# Autodesk Inventor assembly: SEPARACION LATA-BOTELLA Y PAPEL
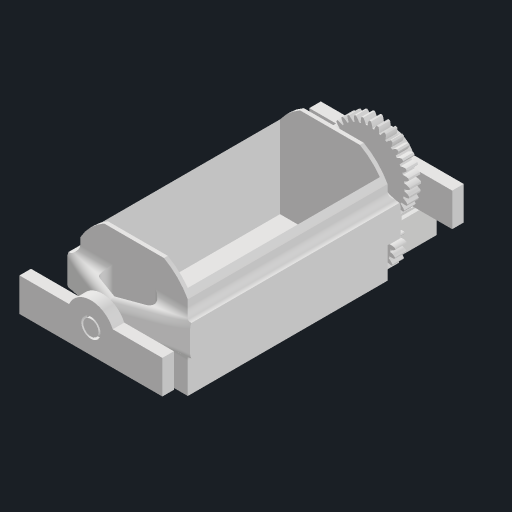
[picture p0: Inventor's stored thumbnail of the model, 512x512]
Saved by Autodesk Inventor 2024.3 (Build 283343000, 343)
## iProperties
Created: 2024-06-16
Part Number: SEPARACION LATA-BOTELLA Y PAPEL
Document SubType Name: Assembly
Designer: Jhuliams
Author: Jhuliams
## Documents named in this file (7)
- C:\Users\Niler\OneDrive\Escritorio\RECICLADOR\RECICLADOR_MODELO_3D\MECANISMO DE COMPACTADO\SEPARACION LATA-BOTELLA Y PAPEL.iam
- C:\Users\Niler\OneDrive\Escritorio\RECICLADOR\RECICLADOR_MODELO_3D\MECANISMO DE COMPACTADO\CAJA PARA DETECCION DE OBJETO.ipt
- C:\Users\Niler\OneDrive\Escritorio\RECICLADOR\RECICLADOR_MODELO_3D\MECANISMO DE COMPACTADO\ENGRANAJE CONDUCTOR DE CAJA.ipt
- C:\Users\Niler\OneDrive\Escritorio\RECICLADOR\RECICLADOR_MODELO_3D\MECANISMO DE COMPACTADO\ENGRANE MOTRIZ DE CAJA.ipt
- C:\Users\Niler\OneDrive\Escritorio\RECICLADOR\RECICLADOR_MODELO_3D\MECANISMO DE COMPACTADO\SOPORTE DE CAJA SEPARADORA.ipt
- C:\Users\Niler\OneDrive\Escritorio\RECICLADOR\RECICLADOR_MODELO_3D\MECANISMO DE COMPACTADO\NEMA 17 PARA TAPA PRINCIPAL.ipt
- C:\Users\Niler\OneDrive\Escritorio\RECICLADOR\RECICLADOR_MODELO_3D\MECANISMO DE COMPACTADO\SOPORTE DE NEMA.ipt
## Components (7 placed, 6 different names)
1. CAJA PARA DETECCION DE OBJETO:1 — Mate:3, Mate:4, Flush:2, Mate:5, Flush:3, Flush:6, Mate:9, Flush:7
2. ENGRANAJE CONDUCTOR DE CAJA:1 — Flush:1, Mate:2, Mate:3, Rotation:1, Mate:9
3. ENGRANE MOTRIZ DE CAJA:1 — Flush:1, Mate:2, Rotation:1, Mate:6, Flush:5
4. SOPORTE DE CAJA SEPARADORA:1 — Mate:5, Flush:3, Flush:6
5. SOPORTE DE CAJA SEPARADORA:2 — Mate:4, Flush:2, Flush:7
6. NEMA 17 PARA TAPA PRINCIPAL:1 — Mate:6, Flush:5, Mate:7, Mate:8, Flush:8
7. SOPORTE DE NEMA:1 — Mate:7, Mate:8, Flush:8
## Relationships (16: Mate 8, Flush 7, RelateRotation 1)
- Flush:1: ENGRANAJE CONDUCTOR DE CAJA:1 ↔ ENGRANE MOTRIZ DE CAJA:1
- Mate:2 (79.5 mm): ENGRANAJE CONDUCTOR DE CAJA:1 ↔ ENGRANE MOTRIZ DE CAJA:1
- Mate:3: CAJA PARA DETECCION DE OBJETO:1 ↔ ENGRANAJE CONDUCTOR DE CAJA:1
- Rotation:1 [RelateRotation] (1.65 ul): ENGRANAJE CONDUCTOR DE CAJA:1 ↔ ENGRANE MOTRIZ DE CAJA:1
- Mate:4: CAJA PARA DETECCION DE OBJETO:1 ↔ SOPORTE DE CAJA SEPARADORA:2
- Flush:2: CAJA PARA DETECCION DE OBJETO:1 ↔ SOPORTE DE CAJA SEPARADORA:2
- Mate:5: CAJA PARA DETECCION DE OBJETO:1 ↔ SOPORTE DE CAJA SEPARADORA:1
- Flush:3: CAJA PARA DETECCION DE OBJETO:1 ↔ SOPORTE DE CAJA SEPARADORA:1
- Mate:6: ENGRANE MOTRIZ DE CAJA:1 ↔ NEMA 17 PARA TAPA PRINCIPAL:1
- Flush:5 (-5 mm): ENGRANE MOTRIZ DE CAJA:1 ↔ NEMA 17 PARA TAPA PRINCIPAL:1
- Flush:6 (39 mm): CAJA PARA DETECCION DE OBJETO:1 ↔ SOPORTE DE CAJA SEPARADORA:1
- Mate:7: NEMA 17 PARA TAPA PRINCIPAL:1 ↔ SOPORTE DE NEMA:1
- Mate:8: NEMA 17 PARA TAPA PRINCIPAL:1 ↔ SOPORTE DE NEMA:1
- Mate:9: CAJA PARA DETECCION DE OBJETO:1 ↔ ENGRANAJE CONDUCTOR DE CAJA:1
- Flush:7 (39 mm): CAJA PARA DETECCION DE OBJETO:1 ↔ SOPORTE DE CAJA SEPARADORA:2
- Flush:8: NEMA 17 PARA TAPA PRINCIPAL:1 ↔ SOPORTE DE NEMA:1
